# Autodesk Inventor assembly: s-assy-link0_light
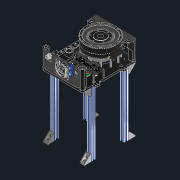
[picture p0: Inventor's stored thumbnail of the model, 180x180]
Saved by Autodesk Inventor 2022 (Build 260153000, 153)
## iProperties
Created: 2021-07-12
Part Number: s-assy-link0_light
Document SubType Name: Assembly
Designer: yuta0
Mass: 7012.56 g
Surface Area: 13530.3 cm^2
Volume: 2705.13 cm^3
Density: 2.59232 g/cm^3
Author: yuta0
## Documents named in this file (19)
- C:\Users\yuta0\Documents\GitHub\catchrobo_hardware\assy-scara\s-assy-link0_light.iam
- C:\Users\yuta0\Documents\GitHub\catchrobo_hardware\assy-scara\alminium_base1.ipt
- C:\Users\yuta0\Documents\GitHub\catchrobo_hardware\assy-scara\CB5-12.ipt
- C:\Users\yuta0\Documents\GitHub\catchrobo_hardware\assy-scara\s-assy-pillar1.iam
- C:\Users\yuta0\Documents\GitHub\catchrobo_hardware\assy-scara\s-assy-pillar2.iam
- C:\Users\yuta0\Documents\GitHub\catchrobo_hardware\assy-scara\s-assy-pillar3.iam
- C:\Users\yuta0\Documents\GitHub\catchrobo_hardware\assy-scara\CB3-5.ipt
- C:\Users\yuta0\Documents\GitHub\catchrobo_hardware\assy-scara\ODrive3.4.ipt
- C:\Users\yuta0\Documents\GitHub\catchrobo_hardware\assy-scara\power_supply_unit.ipt
- C:\Users\yuta0\Documents\GitHub\catchrobo_hardware\assy-scara\U2H-Z7SBK.ipt
- C:\Users\yuta0\Documents\GitHub\catchrobo_hardware\assy-scara\s-assy-unit-j1.iam
- C:\Users\yuta0\Documents\GitHub\catchrobo_hardware\assy-scara\50wr5j cement resistor.ipt
- C:\Users\yuta0\Documents\GitHub\catchrobo_hardware\assy-scara\LBNR3.ipt
- C:\Users\yuta0\Documents\GitHub\catchrobo_hardware\assy-scara\CB4-10.ipt
- C:\Users\yuta0\Documents\GitHub\catchrobo_hardware\assy-scara\hexagonal_spacer_M3_5mm.ipt
- C:\Users\yuta0\Documents\GitHub\catchrobo_hardware\assy-scara\hexagonal_spacer_M3_30mm.ipt
- C:\Users\yuta0\Documents\GitHub\catchrobo_hardware\assy-scara\base46.ipt
- C:\Users\yuta0\Documents\GitHub\catchrobo_hardware\assy-scara\s-assy-base_light.iam
- C:\Users\yuta0\Documents\GitHub\catchrobo_hardware\assy-scara\s-assyypanel_light.iam
## Components (69 placed, 18 different names)
1. alminium_base1:2 — メイト:153, メイト:155, メイト:157, メイト:162, メイト:177, メイト:178, メイト:179, メイト:180, メイト:194, メイト:195, メイト:196, メイト:197, メイト:198, メイト:199, メイト:200, メイト:201, メイト:202, メイト:203, メイト:221, メイト:222, メイト:224, メイト:225, メイト:228, メイト:229, メイト:243, メイト:244, メイト:248, メイト:249, メイト:261
2. s-assy-unit-j1:1 [sub-assembly] — メイト:201, メイト:202, メイト:203, メイト:204, メイト:205, メイト:250, メイト:251, メイト:252
3. s-assy-pillar1:1 [sub-assembly] — メイト:153, メイト:178
4. s-assy-pillar1:2 [sub-assembly] — メイト:155, メイト:179, メイト:181
5. s-assy-pillar2:1 [sub-assembly] — メイト:157, メイト:177, メイト:183, フラッシュ:5, メイト:242
6. s-assy-pillar3:1 [sub-assembly] — メイト:162, メイト:180, メイト:185
7. s-assyypanel_light:1 [sub-assembly] — メイト:182
8. power_supply_unit:1 — メイト:196, メイト:197, メイト:200, メイト:226, メイト:227
9. U2H-Z7SBK:1 — メイト:199, フラッシュ:5
10. 50wr5j cement resistor:3 — メイト:217, メイト:219
11. ODrive3.4:1 — メイト:194, メイト:195, メイト:198, メイト:253, メイト:254
12. LBNR3:2 — メイト:219, メイト:220
13. LBNR3:1 — メイト:217, メイト:218
14. CB3-5:25 — メイト:218
15. CB3-5:26 — メイト:220
16. base46:1 — メイト:250, メイト:251, メイト:252
17. s-assy-base_light:1 [sub-assembly] — メイト:258
18. CB3-5:5
19. CB3-5:6 — メイト:181, メイト:182
20. CB3-5:7
21. CB3-5:8
22. CB3-5:9 — メイト:242
23. CB3-5:10
24. CB3-5:11
25. CB3-5:12
26. CB3-5:13 — メイト:183
27. CB3-5:14 — メイト:185
28. CB3-5:15
29. CB3-5:16
30. CB3-5:17
31. CB3-5:18
32. CB3-5:19
33. CB3-5:20
34. CB3-5:23 — メイト:204, メイト:205
35. CB3-5:24
36. CB4-10:1 — メイト:221, メイト:222
37. CB4-10:2
38. CB4-10:3
39. CB4-10:4
40. CB4-10:5
41. CB4-10:6
42. CB4-10:7
43. CB4-10:8
44. CB4-10:9
45. CB4-10:10
46. CB4-10:11
47. CB4-10:12
48. hexagonal_spacer_M3_5mm:1 — メイト:224, メイト:225, 角度:6
49. CB3-5:31 — メイト:226, メイト:227
50. hexagonal_spacer_M3_5mm:2
51. CB3-5:32
52. hexagonal_spacer_M3_5mm:4
53. CB3-5:34
54. CB5-12:9 — メイト:243, メイト:244
55. CB5-12:10
56. CB5-12:11
57. CB5-12:12 — メイト:258, メイト:261
58. CB3-5:39 — メイト:248, メイト:249
59. CB3-5:40
60. CB3-5:41
61. CB3-5:42
62. CB3-5:35 — メイト:253, メイト:254
63. hexagonal_spacer_M3_30mm:1 — メイト:228, メイト:229, 角度:6
64. CB3-5:43
65. hexagonal_spacer_M3_30mm:2
66. CB3-5:44
67. hexagonal_spacer_M3_30mm:3
68. CB3-5:45
69. hexagonal_spacer_M3_30mm:4
## Component patterns: (4 elements, first: CB3-5:5 + CB3-5:6), (4 elements, first: CB3-5:13 + CB3-5:14), (2 elements, first: CB3-5:23), (12 elements, first: CB4-10:1), (4 elements, first: hexagonal_spacer_M3_5mm:1 + CB3-5:31), (4 elements, first: CB5-12:9), (4 elements, first: CB3-5:39), (4 elements, first: CB3-5:35 + hexagonal_spacer_M3_30mm:1)
## Relationships (50: Mate 48, Flush 1, Angle 1)
- メイト:153 [Mate]: alminium_base1:2 ↔ s-assy-pillar1:1
- メイト:155 [Mate]: alminium_base1:2 ↔ s-assy-pillar1:2
- メイト:157 [Mate]: alminium_base1:2 ↔ s-assy-pillar2:1
- メイト:162 [Mate]: alminium_base1:2 ↔ s-assy-pillar3:1
- メイト:177 [Mate]: alminium_base1:2 ↔ s-assy-pillar2:1
- メイト:178 [Mate]: alminium_base1:2 ↔ s-assy-pillar1:1
- メイト:179 [Mate]: alminium_base1:2 ↔ s-assy-pillar1:2
- メイト:180 [Mate]: alminium_base1:2 ↔ s-assy-pillar3:1
- メイト:181 [Mate]: s-assy-pillar1:2 ↔ CB3-5:6
- メイト:182 [Mate]: s-assyypanel_light:1 ↔ CB3-5:6
- メイト:183 [Mate]: s-assy-pillar2:1 ↔ CB3-5:13
- メイト:185 [Mate]: s-assy-pillar3:1 ↔ CB3-5:14
- メイト:194 [Mate]: alminium_base1:2 ↔ ODrive3.4:1
- メイト:195 [Mate]: alminium_base1:2 ↔ ODrive3.4:1
- メイト:196 [Mate]: alminium_base1:2 ↔ power_supply_unit:1
- メイト:197 [Mate]: alminium_base1:2 ↔ power_supply_unit:1
- メイト:198 [Mate] (30 mm): alminium_base1:2 ↔ ODrive3.4:1
- メイト:199 [Mate]: alminium_base1:2 ↔ U2H-Z7SBK:1
- フラッシュ:5 [Flush]: s-assy-pillar2:1 ↔ U2H-Z7SBK:1
- メイト:200 [Mate] (5 mm): alminium_base1:2 ↔ power_supply_unit:1
- メイト:201 [Mate]: alminium_base1:2 ↔ s-assy-unit-j1:1
- メイト:202 [Mate]: alminium_base1:2 ↔ s-assy-unit-j1:1
- メイト:203 [Mate]: alminium_base1:2 ↔ s-assy-unit-j1:1
- メイト:204 [Mate]: s-assy-unit-j1:1 ↔ CB3-5:23
- メイト:205 [Mate]: s-assy-unit-j1:1 ↔ CB3-5:23
- メイト:217 [Mate]: 50wr5j cement resistor:3 ↔ LBNR3:1
- メイト:218 [Mate]: LBNR3:1 ↔ CB3-5:25
- メイト:219 [Mate]: 50wr5j cement resistor:3 ↔ LBNR3:2
- メイト:220 [Mate]: LBNR3:2 ↔ CB3-5:26
- メイト:221 [Mate]: alminium_base1:2 ↔ CB4-10:1
- メイト:222 [Mate]: alminium_base1:2 ↔ CB4-10:1
- メイト:224 [Mate]: alminium_base1:2 ↔ hexagonal_spacer_M3_5mm:1
- メイト:225 [Mate]: alminium_base1:2 ↔ hexagonal_spacer_M3_5mm:1
- メイト:226 [Mate]: power_supply_unit:1 ↔ CB3-5:31
- メイト:227 [Mate]: power_supply_unit:1 ↔ CB3-5:31
- メイト:228 [Mate]: alminium_base1:2 ↔ hexagonal_spacer_M3_30mm:1
- メイト:229 [Mate]: alminium_base1:2 ↔ hexagonal_spacer_M3_30mm:1
- 角度:6 [Angle] (0 deg): hexagonal_spacer_M3_5mm:1 ↔ hexagonal_spacer_M3_30mm:1
- メイト:242 [Mate]: s-assy-pillar2:1 ↔ CB3-5:9
- メイト:243 [Mate]: alminium_base1:2 ↔ CB5-12:9
- メイト:244 [Mate] (4.5 mm): alminium_base1:2 ↔ CB5-12:9
- メイト:248 [Mate]: alminium_base1:2 ↔ CB3-5:39
- メイト:249 [Mate]: alminium_base1:2 ↔ CB3-5:39
- メイト:250 [Mate]: s-assy-unit-j1:1 ↔ base46:1
- メイト:251 [Mate]: s-assy-unit-j1:1 ↔ base46:1
- メイト:252 [Mate]: s-assy-unit-j1:1 ↔ base46:1
- メイト:253 [Mate]: ODrive3.4:1 ↔ CB3-5:35
- メイト:254 [Mate]: ODrive3.4:1 ↔ CB3-5:35
- メイト:258 [Mate]: s-assy-base_light:1 ↔ CB5-12:12
- メイト:261 [Mate]: alminium_base1:2 ↔ CB5-12:12
